# Autodesk Inventor assembly: A2017_T2_08
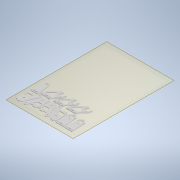
[picture p0: Inventor's stored thumbnail of the model, 180x180]
Saved by Autodesk Inventor 2020 (Build 240168000, 168)
## iProperties
Created: 2021-08-27
Part Number: A2017_T2_08
Document SubType Name: Assembly
Designer: Masato
Author: Masato
## Documents named in this file (6)
- C:\Inventor\SUSTAINA-OP\Cam\A2017_T2_08.iam
- C:\Inventor\SUSTAINA-OP\Cam\DisposableBoard.ipt
- C:\Inventor\SUSTAINA-OP\LowerBody\Leg_joint\Leg_joint_pitch_frame.ipt
- C:\Inventor\SUSTAINA-OP\LowerBody\Foot\Foot_back_frame.ipt
- C:\Inventor\SUSTAINA-OP\LowerBody\Foot\Foot_front_frame.ipt
- C:\Inventor\SUSTAINA-OP\UpperBody\Arm\Shoulder_side_frame.ipt
## Components (11 placed, 5 different names)
1. DisposableBoard:1 — メイト:2, メイト:1, フラッシュ:1, フラッシュ:2, メイト:4, メイト:5, メイト:7, メイト:8, 正接:2, メイト:11, フラッシュ:6, フラッシュ:7, フラッシュ:8, メイト:15, メイト:16, フラッシュ:10
2. Leg_joint_pitch_frame:1 — メイト:5, メイト:9, フラッシュ:7, フラッシュ:8, フラッシュ:9, メイト:17
3. Leg_joint_pitch_frame:2 — メイト:4, メイト:13, フラッシュ:9, メイト:14
4. Leg_joint_pitch_frame:3 — メイト:7, メイト:9, 正接:2, メイト:10, フラッシュ:5, メイト:18
5. Leg_joint_pitch_frame:4 — メイト:8, メイト:10, フラッシュ:5, メイト:13
6. Foot_front_frame:1 — メイト:15, メイト:17, フラッシュ:10, メイト:19
7. Foot_back_frame:1 — メイト:11, フラッシュ:6, メイト:14
8. Foot_back_frame:2
9. Shoulder_side_frame:1 — メイト:16, メイト:18, メイト:19
10. Shoulder_side_frame:2
11. Shoulder_side_frame:3
## Component patterns: (2 elements, first: Foot_back_frame:1), (3 elements, first: Shoulder_side_frame:1)
## Relationships (25: Mate 16, Flush 8, Tangent 1)
- メイト:2 [Mate]: DisposableBoard:1
- メイト:1 [Mate]: DisposableBoard:1
- フラッシュ:1 [Flush]: DisposableBoard:1
- フラッシュ:2 [Flush]: DisposableBoard:1
- メイト:4 [Mate]: DisposableBoard:1 ↔ Leg_joint_pitch_frame:2
- メイト:5 [Mate]: DisposableBoard:1 ↔ Leg_joint_pitch_frame:1
- メイト:7 [Mate]: DisposableBoard:1 ↔ Leg_joint_pitch_frame:3
- メイト:8 [Mate]: DisposableBoard:1 ↔ Leg_joint_pitch_frame:4
- メイト:9 [Mate] (2.5 mm): Leg_joint_pitch_frame:1 ↔ Leg_joint_pitch_frame:3
- 正接:2 [Tangent] (2 mm): DisposableBoard:1 ↔ Leg_joint_pitch_frame:3
- メイト:10 [Mate] (2.5 mm): Leg_joint_pitch_frame:3 ↔ Leg_joint_pitch_frame:4
- フラッシュ:5 [Flush]: Leg_joint_pitch_frame:3 ↔ Leg_joint_pitch_frame:4
- メイト:11 [Mate]: DisposableBoard:1 ↔ Foot_back_frame:1
- フラッシュ:6 [Flush] (2 mm): DisposableBoard:1 ↔ Foot_back_frame:1
- フラッシュ:7 [Flush] (2 mm): DisposableBoard:1 ↔ Leg_joint_pitch_frame:1
- フラッシュ:8 [Flush] (2 mm): DisposableBoard:1 ↔ Leg_joint_pitch_frame:1
- メイト:13 [Mate] (2.5 mm): Leg_joint_pitch_frame:2 ↔ Leg_joint_pitch_frame:4
- フラッシュ:9 [Flush]: Leg_joint_pitch_frame:1 ↔ Leg_joint_pitch_frame:2
- メイト:14 [Mate] (2.5 mm): Leg_joint_pitch_frame:2 ↔ Foot_back_frame:1
- メイト:15 [Mate]: DisposableBoard:1 ↔ Foot_front_frame:1
- メイト:16 [Mate]: DisposableBoard:1 ↔ Shoulder_side_frame:1
- メイト:17 [Mate] (4.5 mm): Leg_joint_pitch_frame:1 ↔ Foot_front_frame:1
- フラッシュ:10 [Flush] (2 mm): DisposableBoard:1 ↔ Foot_front_frame:1
- メイト:18 [Mate] (2.5 mm): Leg_joint_pitch_frame:3 ↔ Shoulder_side_frame:1
- メイト:19 [Mate] (2.5 mm): Foot_front_frame:1 ↔ Shoulder_side_frame:1
